# Autodesk Inventor assembly: Engine Assembly
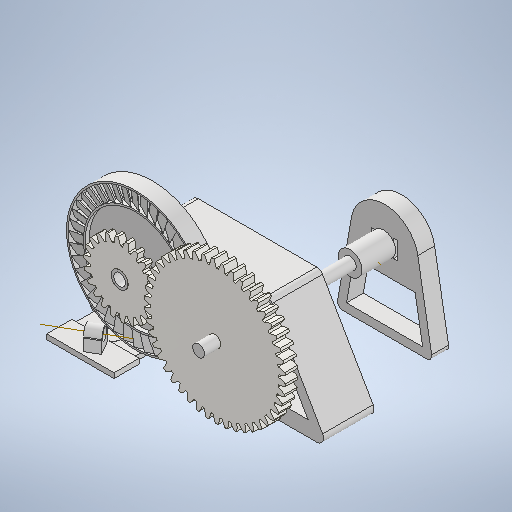
[picture p0: Inventor's stored thumbnail of the model, 512x512]
Saved by Autodesk Inventor 2026.1 (Build 301233020, 233B)
## iProperties
Created: 2025-11-03
Part Number: Engine Assembly
Document SubType Name: Assembly
Designer: yo
Author: yo
## Documents named in this file (8)
- C:\Users\yo\Documents\Andes\9no Semestre\Proyecto Intermedio\Proyecto\Huron-Hudson\Pelton Engine\V10\Engine Assembly.iam
- C:\Users\yo\Documents\Andes\9no Semestre\Proyecto Intermedio\Proyecto\Huron-Hudson\Pelton Engine\V10\EngineMount - Big hole.ipt
- C:\Users\yo\Documents\Andes\9no Semestre\Proyecto Intermedio\Proyecto\Huron-Hudson\Pelton Engine\V10\Impulse Turbine 2.ipt
- C:\Users\yo\Documents\Andes\9no Semestre\Proyecto Intermedio\Proyecto\Huron-Hudson\Pelton Engine\V10\Shaft.ipt
- C:\Users\yo\Documents\Andes\9no Semestre\Proyecto Intermedio\Proyecto\Huron-Hudson\Pelton Engine\V10\Engine Assembly\Design Accelerator\Spur Gears1.iam
- C:\Users\yo\Documents\Andes\9no Semestre\Proyecto Intermedio\Proyecto\Huron-Hudson\Pelton Engine\V10\Sensor Stand.ipt
- C:\Users\yo\Documents\Andes\9no Semestre\Proyecto Intermedio\Proyecto\Huron-Hudson\Pelton Engine\V10\Magnet Coupler.ipt
- C:\Users\yo\Documents\Andes\9no Semestre\Proyecto Intermedio\Proyecto\Huron-Hudson\Pelton Engine\V10\Nozzle Fixer.ipt
## Components (7 placed, 7 different names)
1. EngineMount - Big hole:1 — Flush:1, Flush:2, Flush:3, Mate:1, Tangent:1, Mate:2, Tangent:2, Mate:11, Flush:6
2. Impulse Turbine 2:1 — Mate:1, Tangent:1, Mate:3, Mate:4, Mate:6
3. Shaft:1 — Mate:2, Flush:4, Mate:5, Mate:7, Mate:8, Mate:9, Rotation:1, Rotation:2
4. Spur Gears:1 [sub-assembly] — Mate:3, Mate:4, Mate:5, Mate:6, Rotation:2
5. Sensor Stand:1 — Mate:7, Flush:5, Mate:10
6. Magnet Coupler:1 — Mate:8, Mate:9, Rotation:1, Mate:10
7. Nozzle Fixer:1 — Tangent:2, Mate:11, Flush:6, Mate:12
## Relationships (22: Mate 12, Flush 6, Tangent 2, RelateRotation 2)
- Flush:1: EngineMount - Big hole:1
- Flush:2: EngineMount - Big hole:1
- Flush:3: EngineMount - Big hole:1
- Mate:1: EngineMount - Big hole:1 ↔ Impulse Turbine 2:1
- Tangent:1: EngineMount - Big hole:1 ↔ Impulse Turbine 2:1
- Mate:2: EngineMount - Big hole:1 ↔ Shaft:1
- Flush:4: Shaft:1
- Mate:3: Impulse Turbine 2:1 ↔ Spur Gears:1
- Mate:4: Impulse Turbine 2:1 ↔ Spur Gears:1
- Mate:5: Shaft:1 ↔ Spur Gears:1
- Mate:6: Impulse Turbine 2:1 ↔ Spur Gears:1
- Mate:7: Shaft:1 ↔ Sensor Stand:1
- Flush:5: Sensor Stand:1
- Mate:8: Shaft:1 ↔ Magnet Coupler:1
- Mate:9: Shaft:1 ↔ Magnet Coupler:1
- Rotation:1 [RelateRotation] (1 ul): Shaft:1 ↔ Magnet Coupler:1
- Rotation:2 [RelateRotation] (1 ul): Shaft:1 ↔ Spur Gears:1
- Mate:10 (0.5 mm): Sensor Stand:1 ↔ Magnet Coupler:1
- Tangent:2: EngineMount - Big hole:1 ↔ Nozzle Fixer:1
- Mate:11: EngineMount - Big hole:1 ↔ Nozzle Fixer:1
- Flush:6: EngineMount - Big hole:1 ↔ Nozzle Fixer:1
- Mate:12: Nozzle Fixer:1
